# Autodesk Inventor assembly: Solids Feeder Head Assembly
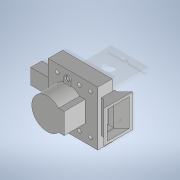
[picture p0: Inventor's stored thumbnail of the model, 180x180]
Saved by Autodesk Inventor 2022 (Build 260153000, 153)
## iProperties
Created: 2022-04-23
Part Number: Solids Feeder Head Assembly
Document SubType Name: Assembly
Designer: efred
Author: efred
## Documents named in this file (7)
- C:\Users\efred\OneDrive - Imperial College London\Old Shit\ROBOICP\Final Assembly\Solids Feeder Head Assembly.iam
- C:\Users\efred\OneDrive - Imperial College London\Old Shit\ROBOICP\Final Assembly\paddle rotor.ipt
- C:\Users\efred\OneDrive - Imperial College London\Old Shit\ROBOICP\Final Assembly\smol stepper.ipt
- C:\Users\efred\OneDrive - Imperial College London\Old Shit\ROBOICP\Final Assembly\body.ipt
- C:\Users\efred\OneDrive - Imperial College London\Old Shit\ROBOICP\Final Assembly\body cover.ipt
- C:\Users\efred\OneDrive - Imperial College London\Old Shit\ROBOICP\Final Assembly\solids hopper.ipt
- C:\Users\efred\OneDrive - Imperial College London\Old Shit\ROBOICP\Final Assembly\hopper lid.ipt
## Components (6 placed, 6 different names)
1. paddle rotor:1 — Mate:1, Mate:2, Flush:5, Flush:6
2. smol stepper:1 — Mate:1, Mate:2, Flush:1, Flush:4
3. body:1 — Flush:2, Flush:3, Flush:4, Flush:5, Flush:6, Flush:7, Flush:10, Flush:11
4. body cover:1 — Flush:8, Flush:9
5. solids hopper:1 — Flush:10, Flush:11, Flush:12, Flush:14
6. hopper lid:1 — Flush:13
## Relationships (16: Flush 14, Mate 2)
- Mate:1 (0.1 mm): paddle rotor:1 ↔ smol stepper:1
- Mate:2: paddle rotor:1 ↔ smol stepper:1
- Flush:1 (0.1 mm): smol stepper:1
- Flush:2: body:1
- Flush:3: body:1
- Flush:4 (0.1 mm): smol stepper:1 ↔ body:1
- Flush:5 (0.1 mm): paddle rotor:1 ↔ body:1
- Flush:6 (0.1 mm): paddle rotor:1 ↔ body:1
- Flush:7 (0.1 mm): body:1
- Flush:8: body cover:1
- Flush:9: body cover:1
- Flush:10: body:1 ↔ solids hopper:1
- Flush:11 (0.1 mm): body:1 ↔ solids hopper:1
- Flush:12 (0.1 mm): solids hopper:1
- Flush:13: hopper lid:1
- Flush:14 (0.1 mm): solids hopper:1
